# Autodesk Inventor assembly: V-Wheel Solid Wheel
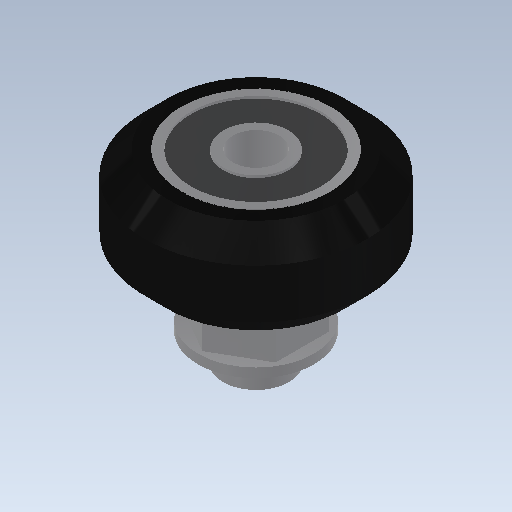
[picture p0: Inventor's stored thumbnail of the model, 512x512]
Saved by Autodesk Inventor 2020.3 (Build 243373000, 373)
## iProperties
Created: 2016-04-10
Part Number: V-Wheel Solid Wheel
Document SubType Name: Assembly
Designer: Ben
Mass: 4.36888 g
Surface Area: 37.8181 cm^2
Volume: 4.36888 cm^3
Density: 1 g/cm^3
Author: Ben
## Documents named in this file (5)
- C:\Users\juanp\Desktop\Robocol\Diseño EVA\Actuador Lineal\Placas deslizantes\V-Wheel Solid Wheel.iam
- C:\Users\juanp\Desktop\Robocol\Diseño EVA\Actuador Lineal\Placas deslizantes\Solid V-Wheel.ipt
- C:\Users\juanp\Desktop\Robocol\Diseño EVA\Actuador Lineal\Placas deslizantes\Ball Bearing 625 2RS 5x16x5.ipt
- C:\Users\juanp\Desktop\Robocol\Diseño EVA\Actuador Lineal\Placas deslizantes\Eccentric Spacer.ipt
- C:\Users\juanp\Desktop\Robocol\Diseño EVA\Actuador Lineal\Placas deslizantes\1mm 5mm shim.ipt
## Components (5 placed, 4 different names)
1. Solid V-Wheel:1 — Mate:1, Mate:2, Flush:1
2. Ball Bearing 625 2RS 5x16x5:1 — Mate:1, Mate:3, Mate:4, Mate:5, Mate:7
3. Ball Bearing 625 2RS 5x16x5:2 — Mate:2, Mate:3, Flush:1
4. Eccentric Spacer:1 — Mate:6, Mate:7
5. 1mm 5mm shim:1 — Mate:4, Mate:5, Mate:6
## Relationships (8: Mate 7, Flush 1)
- Mate:1: Solid V-Wheel:1 ↔ Ball Bearing 625 2RS 5x16x5:1
- Mate:2: Solid V-Wheel:1 ↔ Ball Bearing 625 2RS 5x16x5:2
- Mate:3: Ball Bearing 625 2RS 5x16x5:1 ↔ Ball Bearing 625 2RS 5x16x5:2
- Flush:1: Solid V-Wheel:1 ↔ Ball Bearing 625 2RS 5x16x5:2
- Mate:4: Ball Bearing 625 2RS 5x16x5:1 ↔ 1mm 5mm shim:1
- Mate:5: Ball Bearing 625 2RS 5x16x5:1 ↔ 1mm 5mm shim:1
- Mate:6: Eccentric Spacer:1 ↔ 1mm 5mm shim:1
- Mate:7: Ball Bearing 625 2RS 5x16x5:1 ↔ Eccentric Spacer:1
